# Autodesk Inventor assembly: disc Aero arm fit check
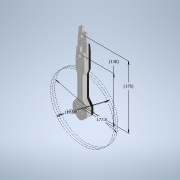
[picture p0: Inventor's stored thumbnail of the model, 180x180]
Saved by Autodesk Inventor 2020 (Build 240168000, 168)
## iProperties
Created: 2022-06-23
Part Number: disc Aero arm fit check
Document SubType Name: Assembly
Designer: Steven
Author: Steven
## Documents named in this file (5)
- Y:\FPV drone stuff\0 Street League\Frames\experimental-quad-frames\disc Aero arm fit check.iam
- Y:\FPV drone stuff\0 Street League\Frames\PB-Kauri-X\Kauri arm.ipt
- Y:\FPV drone stuff\0 Street League\Frames\experimental-quad-frames\Kauri arm disc aero.ipt
- Y:\FPV drone stuff\0 Street League\Frames\experimental-quad-frames\Kauri arm long disc aero.ipt
- Y:\FPV drone stuff\0 Street League\Frames\experimental-quad-frames\Kauri arm short disc aero.ipt
## Components (4 placed, 4 different names)
1. Kauri arm:1 — Mate:1, Flush:1, Flush:2, Flush:3, Mate:2, Mate:3, Mate:4, Mate:6
2. Kauri arm disc aero:1 — Mate:1, Mate:2, Mate:3, Mate:4, Mate:5, Mate:8
3. Kauri arm long disc aero:1 — Mate:5, Mate:6, Mate:7
4. Kauri arm short disc aero:1 — Mate:7, Mate:8
## Relationships (11: Mate 8, Flush 3)
- Mate:1: Kauri arm:1 ↔ Kauri arm disc aero:1
- Flush:1: Kauri arm:1
- Flush:2: Kauri arm:1
- Flush:3: Kauri arm:1
- Mate:2: Kauri arm:1 ↔ Kauri arm disc aero:1
- Mate:3: Kauri arm:1 ↔ Kauri arm disc aero:1
- Mate:4: Kauri arm:1 ↔ Kauri arm disc aero:1
- Mate:5: Kauri arm disc aero:1 ↔ Kauri arm long disc aero:1
- Mate:6: Kauri arm:1 ↔ Kauri arm long disc aero:1
- Mate:7: Kauri arm long disc aero:1 ↔ Kauri arm short disc aero:1
- Mate:8: Kauri arm disc aero:1 ↔ Kauri arm short disc aero:1
